# Autodesk Inventor assembly: Shaft_Sprocket_Assembly
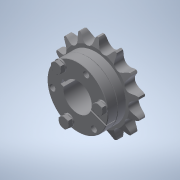
[picture p0: Inventor's stored thumbnail of the model, 180x180]
Saved by Autodesk Inventor 2021 (Build 250183000, 183)
## iProperties
Created: 2020-10-13
Part Number: Shaft_Sprocket_Assembly
Document SubType Name: Assembly
Designer: PhotonUser
Quantity: 1
Author: PhotonUser
## Documents named in this file (3)
- D:\PhotonUser\Downloads\Assembly Files-20201111T001656Z-001\Assembly Files\Shaft_Sprocket_Assembly.iam
- D:\PhotonUser\Downloads\Assembly Files-20201111T001656Z-001\Assembly Files\6086K221_QUICK-DISCONNECT BUSHING.ipt
- D:\PhotonUser\Downloads\Assembly Files-20201111T001656Z-001\Assembly Files\62375K141_QUICK-DISCONNECT BUSHING-BORE SPROCKET.ipt
## Components (2 placed, 2 different names)
1. 6086K221_QUICK-DISCONNECT BUSHING:1 — Insert:1, Insert:2
2. 62375K141_QUICK-DISCONNECT BUSHING-BORE SPROCKET:1 — Insert:1, Insert:2
## Relationships (2: Insert 2)
- Insert:1: 6086K221_QUICK-DISCONNECT BUSHING:1 ↔ 62375K141_QUICK-DISCONNECT BUSHING-BORE SPROCKET:1
- Insert:2: 6086K221_QUICK-DISCONNECT BUSHING:1 ↔ 62375K141_QUICK-DISCONNECT BUSHING-BORE SPROCKET:1
